# Autodesk Inventor assembly: 2024_0222_OmniC
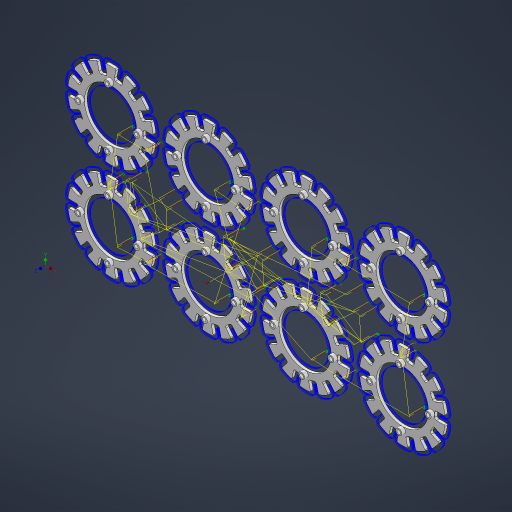
[picture p0: Inventor's stored thumbnail of the model, 512x512]
Saved by Autodesk Inventor 2024.2 (Build 282272000, 272)
## iProperties
Created: 2024-02-22
Part Number: 2024_0222_OmniC
Document SubType Name: Assembly
Designer: Hanaoka
Author: Hanaoka
## Documents named in this file (2)
- G:\共有ドライブ\reRo\05_個人\hanaoka\inventor\CAMpath\2024_0222_OmniC.iam
- G:\共有ドライブ\reRo\05_個人\hanaoka\inventor\DriveUnit\OmniFrame_C.ipt
## Components (8 placed, 1 different names)
1. OmniFrame_C:1 — メイト:1, メイト:2, 正接:1
2. OmniFrame_C:2
3. OmniFrame_C:3
4. OmniFrame_C:4
5. OmniFrame_C:5
6. OmniFrame_C:6
7. OmniFrame_C:7
8. OmniFrame_C:8
## Component patterns: (8 elements, first: OmniFrame_C:1)
## Relationships (3: Mate 2, Tangent 1)
- メイト:1 [Mate]: OmniFrame_C:1
- メイト:2 [Mate] (6 mm): OmniFrame_C:1
- 正接:1 [Tangent]: OmniFrame_C:1
